# Autodesk Inventor assembly: beanintake
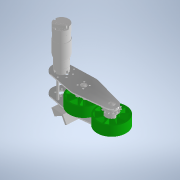
[picture p0: Inventor's stored thumbnail of the model, 180x180]
Saved by Autodesk Inventor 2020 (Build 240168000, 168)
## iProperties
Created: 2019-12-28
Part Number: beanintake
Document SubType Name: Assembly
Designer: xj82b
Author: xj82b
## Documents named in this file (14)
- C:\Users\xj82b\Documents\Inventor\5199\beanintake.iam
- C:\Users\xj82b\Documents\Inventor\5199\bean.ipt
- C:\Users\xj82b\Documents\Inventor\5199\gobilda parts\1501-0006-0480.ipt
- C:\Users\xj82b\Documents\Inventor\5199\andymark parts\am-3946 3IN 375Hex Compliant Wheel VER 3.ipt
- C:\Users\xj82b\Documents\Inventor\5199\gobilda parts\5202-0002-0005 part.ipt
- C:\Users\xj82b\Documents\Inventor\5199\gobilda parts\1611-0514-0006.ipt
- C:\Users\xj82b\Documents\Inventor\5199\pressfit.ipt
- C:\Users\xj82b\Documents\Inventor\5199\gobilda parts\2101-0006-0060.ipt
- C:\Users\xj82b\Documents\Inventor\5199\gobilda parts\1309-0016-1006 assembly.ipt
- C:\Users\xj82b\Documents\Inventor\5199\gobilda parts\3310-0014-0014.ipt
- C:\Users\xj82b\Documents\Inventor\5199\gobilda parts\1500-0010-0006.ipt
- C:\Users\xj82b\Documents\Inventor\5199\9.6 spacer.ipt
- C:\Users\xj82b\Documents\Inventor\5199\gobilda parts\1608-0001-0001 assembly.ipt
- C:\Users\xj82b\Documents\Inventor\5199\intakemount.ipt
## Components (25 placed, 13 different names)
1. bean:1 — Mate:1, Mate:4, Mate:7, Mate:8, Mate:25, Mate:26, Mate:54, Mate:55, Mate:59, Mate:64
2. bean:2 — Mate:9, Mate:11, Mate:12, Mate:13, Mate:14, Mate:23, Mate:24, Flush:2, Mate:52, Mate:53, Flush:3
3. 1501-0006-0480:1 — Mate:1, Mate:7, Mate:9
4. 1501-0006-0480:3 — Mate:4, Mate:8, Mate:11
5. am-3946 3IN 375Hex Compliant Wheel VER 3:1 — Mate:19, Mate:20, Flush:1, Mate:32
6. 5202-0002-0005 part:1 — Mate:12, Mate:13, Mate:14
7. pressfit:1 — Mate:19, Mate:20, Flush:1, Mate:21, Mate:22, Mate:37
8. 2101-0006-0060:1 — Mate:21, Mate:22, Mate:27, Mate:31, Flush:2
9. 1611-0514-0006:3 — Mate:23, Mate:24, Mate:38, Mate:58
10. 1611-0514-0006:4 — Mate:25, Mate:26, Mate:27, Mate:35, Mate:36
11. 1309-0016-1006 assembly:1 — Mate:28, Mate:29, Mate:30, Mate:31, Mate:32, Mate:39
12. 3310-0014-0014:1 — Mate:28, Mate:29, Mate:30
13. 1500-0010-0006:2 — Mate:35, Mate:36, Mate:37
14. 9.6 spacer:1 — Mate:38, Mate:39, Mate:58
15. pressfit:2 — Mate:45, Mate:46, Mate:47, Mate:48, Mate:50
16. 1309-0016-1006 assembly:2 — Mate:49
17. 3310-0014-0014:2
18. 1500-0010-0006:3 — Mate:45
19. 9.6 spacer:2 — Mate:51, Mate:56, Mate:57
20. am-3946 3IN 375Hex Compliant Wheel VER 3:2 — Mate:46, Mate:47, Mate:48, Mate:49
21. 2101-0006-0060:2 — Mate:50, Mate:51, Flush:3
22. 1611-0514-0006:5 — Mate:52, Mate:53, Mate:56, Mate:57
23. 1611-0514-0006:6 — Mate:54, Mate:55
24. 1608-0001-0001 assembly:1 — Mate:59, Mate:61, Mate:62, Mate:63, Mate:64
25. intakemount:1 — Mate:61, Mate:62, Mate:63
## Relationships (55: Mate 52, Flush 3)
- Mate:1: bean:1 ↔ 1501-0006-0480:1
- Mate:4: bean:1 ↔ 1501-0006-0480:3
- Mate:7: bean:1 ↔ 1501-0006-0480:1
- Mate:8: bean:1 ↔ 1501-0006-0480:3
- Mate:9: bean:2 ↔ 1501-0006-0480:1
- Mate:11: bean:2 ↔ 1501-0006-0480:3
- Mate:12: bean:2 ↔ 5202-0002-0005 part:1
- Mate:13: bean:2 ↔ 5202-0002-0005 part:1
- Mate:14: bean:2 ↔ 5202-0002-0005 part:1
- Mate:19: am-3946 3IN 375Hex Compliant Wheel VER 3:1 ↔ pressfit:1
- Mate:20: am-3946 3IN 375Hex Compliant Wheel VER 3:1 ↔ pressfit:1
- Flush:1: am-3946 3IN 375Hex Compliant Wheel VER 3:1 ↔ pressfit:1
- Mate:21: pressfit:1 ↔ 2101-0006-0060:1
- Mate:22: pressfit:1 ↔ 2101-0006-0060:1
- Mate:23: bean:2 ↔ 1611-0514-0006:3
- Mate:24: bean:2 ↔ 1611-0514-0006:3
- Mate:25: bean:1 ↔ 1611-0514-0006:4
- Mate:26: bean:1 ↔ 1611-0514-0006:4
- Mate:27: 2101-0006-0060:1 ↔ 1611-0514-0006:4
- Mate:28: 1309-0016-1006 assembly:1 ↔ 3310-0014-0014:1
- Mate:29: 1309-0016-1006 assembly:1 ↔ 3310-0014-0014:1
- Mate:30: 1309-0016-1006 assembly:1 ↔ 3310-0014-0014:1
- Mate:31: 2101-0006-0060:1 ↔ 1309-0016-1006 assembly:1
- Mate:32: am-3946 3IN 375Hex Compliant Wheel VER 3:1 ↔ 1309-0016-1006 assembly:1
- Mate:35: 1611-0514-0006:4 ↔ 1500-0010-0006:2
- Mate:36: 1611-0514-0006:4 ↔ 1500-0010-0006:2
- Mate:37: pressfit:1 ↔ 1500-0010-0006:2
- Mate:38: 1611-0514-0006:3 ↔ 9.6 spacer:1
- Mate:39: 1309-0016-1006 assembly:1 ↔ 9.6 spacer:1
- Flush:2 (-2.5 mm): bean:2 ↔ 2101-0006-0060:1
- [Mate]: 1309-0016-1006 assembly:2 ↔ 3310-0014-0014:2
- [Mate]: 1309-0016-1006 assembly:2 ↔ 3310-0014-0014:2
- [Mate]: 1309-0016-1006 assembly:2 ↔ 3310-0014-0014:2
- [Mate]: pressfit:2 ↔ 1500-0010-0006:3
- [Mate]: 1309-0016-1006 assembly:2 ↔ 9.6 spacer:2
- Mate:45: pressfit:2 ↔ 1500-0010-0006:3
- Mate:46: pressfit:2 ↔ am-3946 3IN 375Hex Compliant Wheel VER 3:2
- Mate:47: pressfit:2 ↔ am-3946 3IN 375Hex Compliant Wheel VER 3:2
- Mate:48: pressfit:2 ↔ am-3946 3IN 375Hex Compliant Wheel VER 3:2
- Mate:49: 1309-0016-1006 assembly:2 ↔ am-3946 3IN 375Hex Compliant Wheel VER 3:2
- Mate:50: pressfit:2 ↔ 2101-0006-0060:2
- Mate:51: 9.6 spacer:2 ↔ 2101-0006-0060:2
- Mate:52: bean:2 ↔ 1611-0514-0006:5
- Mate:53: bean:2 ↔ 1611-0514-0006:5
- Mate:54: bean:1 ↔ 1611-0514-0006:6
- Mate:55: bean:1 ↔ 1611-0514-0006:6
- Mate:56: 9.6 spacer:2 ↔ 1611-0514-0006:5
- Mate:57: 9.6 spacer:2 ↔ 1611-0514-0006:5
- Flush:3 (-2.5 mm): bean:2 ↔ 2101-0006-0060:2
- Mate:58: 1611-0514-0006:3 ↔ 9.6 spacer:1
- Mate:59: bean:1 ↔ 1608-0001-0001 assembly:1
- Mate:61: 1608-0001-0001 assembly:1 ↔ intakemount:1
- Mate:62: 1608-0001-0001 assembly:1 ↔ intakemount:1
- Mate:63: 1608-0001-0001 assembly:1 ↔ intakemount:1
- Mate:64: bean:1 ↔ 1608-0001-0001 assembly:1
## Named parameters: d56_d54 = 0 mm, d57_d42 = 0 mm, d58_d43 = 0 mm, d59_d44 = 0 mm, d60_d52 = 0 mm
